# Autodesk Inventor assembly: MIRleft脚一枚
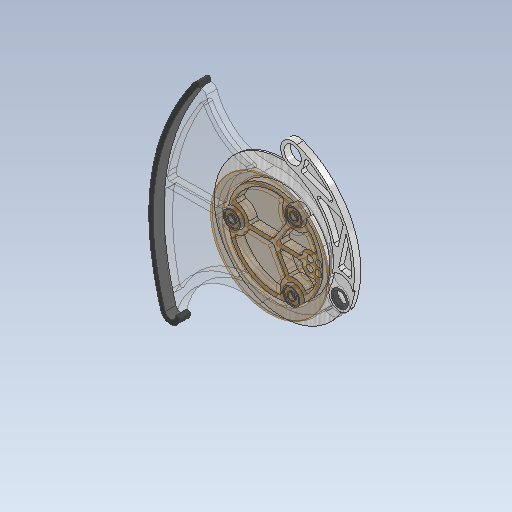
[picture p0: Inventor's stored thumbnail of the model, 512x512]
Saved by Autodesk Inventor 2020.2 (Build 242310000, 310)
## iProperties
Created: 2020-04-13
Part Number: MIRleft脚一枚
Document SubType Name: Assembly
Designer: aoyama
Mass: 31.6013 g
Surface Area: 259.988 cm^2
Volume: 17.8864 cm^3
Density: 1.76678 g/cm^3
Author: aoyama
## Documents named in this file (8)
- C:\Users\aoyam\Desktop\SRDC_local\Inventor\二年機\Geminiβ\脚\ネジクランク\MIR達\MIRleft脚一枚.iam
- C:\Users\aoyam\Desktop\SRDC_local\Inventor\二年機\Geminiβ\脚\ネジクランク\MIR達\MIRleftクランク3t.ipt
- C:\Users\aoyam\Desktop\SRDC_local\Inventor\二年機\Geminiβ\脚\ネジクランク\MIR達\MIRleftクランク4t.ipt
- C:\Users\aoyam\Desktop\SRDC_local\Inventor\二年機\Geminiβ\汎用部品\MIR達\MIRleftベアリングd3D8B4F無.ipt
- C:\Users\aoyam\Desktop\SRDC_local\Inventor\二年機\Geminiβ\脚\ネジクランク\MIR達\MIRleftヘッケン改.ipt
- C:\Users\aoyam\Desktop\SRDC_local\Inventor\二年機\Geminiβ\脚\ネジクランク\MIR達\MIRleft揺動節.ipt
- C:\Users\aoyam\Desktop\SRDC_local\Inventor\二年機\Geminiβ\汎用部品\MIR達\MIRleftオイレス外径8内径6L2.ipt
- C:\Users\aoyam\Desktop\SRDC_local\Inventor\二年機\Geminiβ\脚\ネジクランク\MIR達\MIRleft脚ゴム.ipt
## Components (9 placed, 7 different names)
1. MIRleftクランク3t:1 — 挿入:16, 挿入:15, 挿入:17
2. MIRleftクランク4t:1 — 挿入:16, 挿入:14, 挿入:13, 挿入:12
3. MIRleftベアリングd3D8B4F無:1 — 挿入:14
4. MIRleftベアリングd3D8B4F無:2 — 挿入:15, 挿入:13
5. MIRleftベアリングd3D8B4F無:3 — 挿入:12
6. MIRleftヘッケン改:1 — 挿入:17, 挿入:11, 挿入:8, 挿入:18, 挿入:9
7. MIRleft揺動節:1 — 挿入:11
8. MIRleftオイレス外径8内径6L2:1 — 挿入:8
9. MIRleft脚ゴム:1 — 挿入:18, 挿入:9
## Relationships (10: Insert 10)
- 挿入:16 [Insert]: MIRleftクランク3t:1 ↔ MIRleftクランク4t:1
- 挿入:14 [Insert]: MIRleftクランク4t:1 ↔ MIRleftベアリングd3D8B4F無:1
- 挿入:15 [Insert]: MIRleftクランク3t:1 ↔ MIRleftベアリングd3D8B4F無:2
- 挿入:13 [Insert]: MIRleftクランク4t:1 ↔ MIRleftベアリングd3D8B4F無:2
- 挿入:12 [Insert]: MIRleftクランク4t:1 ↔ MIRleftベアリングd3D8B4F無:3
- 挿入:17 [Insert] (0.2 mm): MIRleftクランク3t:1 ↔ MIRleftヘッケン改:1
- 挿入:11 [Insert]: MIRleftヘッケン改:1 ↔ MIRleft揺動節:1
- 挿入:8 [Insert]: MIRleftヘッケン改:1 ↔ MIRleftオイレス外径8内径6L2:1
- 挿入:18 [Insert]: MIRleftヘッケン改:1 ↔ MIRleft脚ゴム:1
- 挿入:9 [Insert]: MIRleftヘッケン改:1 ↔ MIRleft脚ゴム:1
